# Autodesk Inventor assembly: Overview
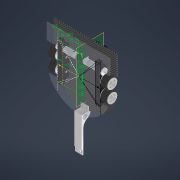
[picture p0: Inventor's stored thumbnail of the model, 180x180]
Saved by Autodesk Inventor 2022 (Build 260153000, 153)
## iProperties
Created: 2021-10-05
Part Number: Overview
Document SubType Name: Assembly
Designer: shiok
Mass: 103.359 g
Surface Area: 978.929 cm^2
Volume: 78.8399 cm^3
Density: 1.311 g/cm^3
Author: shiok
## Documents named in this file (6)
- C:\Users\shiok\Documents\GitHub\murakumo\inventor\Overview.iam
- C:\Users\shiok\Documents\GitHub\murakumo\inventor\flame.ipt
- C:\Users\shiok\Documents\GitHub\murakumo\inventor\Motor.iam
- C:\Users\shiok\Documents\GitHub\murakumo\inventor\Motor_MIR1.iam
- C:\Users\shiok\Documents\GitHub\murakumo\inventor\top.ipt
- C:\Users\shiok\Documents\GitHub\murakumo\inventor\sensorbar.ipt
## Components (5 placed, 5 different names)
1. flame:1 — 挿入:1, 挿入:2
2. Motor:1 [sub-assembly] — 挿入:1
3. Motor_MIR1:1 [sub-assembly] — メイト:1, フラッシュ:2, メイト:3, 挿入:2
4. top:1 — フラッシュ:2, メイト:3, 挿入:3, 挿入:4
5. sensorbar:1 — 挿入:3, 挿入:4
## Relationships (7: Insert 4, Mate 2, Flush 1)
- メイト:1 [Mate] (-42.5 mm): Motor_MIR1:1
- フラッシュ:2 [Flush]: Motor_MIR1:1 ↔ top:1
- メイト:3 [Mate]: Motor_MIR1:1 ↔ top:1
- 挿入:1 [Insert]: flame:1 ↔ Motor:1
- 挿入:2 [Insert]: flame:1 ↔ Motor_MIR1:1
- 挿入:3 [Insert]: top:1 ↔ sensorbar:1
- 挿入:4 [Insert]: top:1 ↔ sensorbar:1
